# Autodesk Inventor assembly: Fan
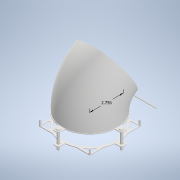
[picture p0: Inventor's stored thumbnail of the model, 180x180]
Saved by Autodesk Inventor 2020 (Build 240168000, 168)
## iProperties
Created: 2020-05-28
Part Number: Fan
Document SubType Name: Assembly
Designer: maple
Author: maple
## Documents named in this file (5)
- C:\Nitro\Github\Air-Conditioner\Air_Conditioner\SubParts\3D\Fan.iam
- C:\Nitro\Github\Air-Conditioner\Air_Conditioner\SubParts\3D\Fan_Part1.ipt
- C:\Nitro\Github\Air-Conditioner\Air_Conditioner\SubParts\3D\Fan_Part2.ipt
- C:\Nitro\Github\Air-Conditioner\Air_Conditioner\SubParts\3D\Fan_Pin.ipt
- C:\Nitro\Github\Air-Conditioner\Air_Conditioner\SubParts\3D\Fan_Part3.ipt
## Components (7 placed, 4 different names)
1. Fan_Part1:1 — Mate:1, Mate:2, Mate:3, Mate:5, Mate:7, Mate:9, Mate:11
2. Fan_Part2:1 — Mate:1, Mate:2, Mate:3, Mate:4, Mate:6, Mate:8, Mate:10, Mate:12
3. Fan_Pin:1 — Mate:4, Mate:5
4. Fan_Pin:2 — Mate:10, Mate:11
5. Fan_Pin:3 — Mate:6, Mate:7
6. Fan_Pin:4 — Mate:8, Mate:9
7. Fan_Part3:1 — Mate:12
## Relationships (12: Mate 12)
- Mate:1 (25 mm): Fan_Part1:1 ↔ Fan_Part2:1
- Mate:2 (25 mm): Fan_Part1:1 ↔ Fan_Part2:1
- Mate:3 (25 mm): Fan_Part1:1 ↔ Fan_Part2:1
- Mate:4: Fan_Part2:1 ↔ Fan_Pin:1
- Mate:5: Fan_Part1:1 ↔ Fan_Pin:1
- Mate:6: Fan_Part2:1 ↔ Fan_Pin:3
- Mate:7: Fan_Part1:1 ↔ Fan_Pin:3
- Mate:8: Fan_Part2:1 ↔ Fan_Pin:4
- Mate:9: Fan_Part1:1 ↔ Fan_Pin:4
- Mate:10: Fan_Part2:1 ↔ Fan_Pin:2
- Mate:11: Fan_Part1:1 ↔ Fan_Pin:2
- Mate:12: Fan_Part2:1 ↔ Fan_Part3:1
